# Autodesk Inventor assembly: splashFurringBase
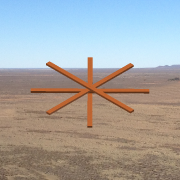
[picture p0: Inventor's stored thumbnail of the model, 180x180]
Saved by Autodesk Inventor 2014 SP1 (Build 180222100, 222)
## iProperties
Created: 2014-05-01
Part Number: splashFurringBase
Document SubType Name: Assembly
Designer: Dave
Author: Dave
## Documents named in this file (2)
- C:\Users\Dave\Desktop\hera-cad\surface\splashFurringBase.iam
- C:\Users\Dave\Desktop\hera-cad\surface\splashFurring.ipt
## Components (4 placed, 1 different names)
1. splashFurring:1 — Insert:1
2. splashFurring:2 — Insert:1, Insert:2
3. splashFurring:3 — Insert:2, Insert:3
4. splashFurring:4 — Insert:3
## Relationships (3: Insert 3)
- Insert:1: splashFurring:1 ↔ splashFurring:2
- Insert:2: splashFurring:2 ↔ splashFurring:3
- Insert:3: splashFurring:3 ↔ splashFurring:4
